# Autodesk Inventor assembly: componentStack
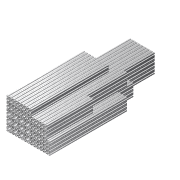
[picture p0: Inventor's stored thumbnail of the model, 180x180]
Saved by Autodesk Inventor 2018 (Build 220112000, 112)
## iProperties
Created: 2018-01-08
Part Number: componentStack
Document SubType Name: Assembly
Designer: sawaiz
Author: sawaiz
## Documents named in this file (7)
- C:\Users\sawaiz\OneDrive\personal\berlin\Move\larkspur\kitchen\frame\extrusions\componentStack.iam
- C:\Users\sawaiz\OneDrive\personal\berlin\Move\larkspur\kitchen\frame\extrusions\HFS5-4040-800.ipt
- C:\Users\sawaiz\OneDrive\personal\berlin\Move\larkspur\kitchen\frame\extrusions\HFS5-2040-500.ipt
- C:\Users\sawaiz\OneDrive\personal\berlin\Move\larkspur\kitchen\frame\extrusions\HFS5-2040-600.ipt
- C:\Users\sawaiz\OneDrive\personal\berlin\Move\larkspur\kitchen\frame\extrusions\HFS5-2020-500.ipt
- C:\Users\sawaiz\OneDrive\personal\berlin\Move\larkspur\kitchen\frame\extrusions\HFS5-2040-560.ipt
- C:\Users\sawaiz\OneDrive\personal\berlin\Move\larkspur\kitchen\frame\extrusions\HFS5-2040-300.ipt
## Components (56 placed, 6 different names)
1. HFS5-4040-800:1 — Flush:2, Mate:3, Flush:5, Flush:6
2. HFS5-4040-800:2
3. HFS5-4040-800:3 — Mate:1
4. HFS5-4040-800:4
5. HFS5-4040-800:5
6. HFS5-4040-800:6
7. HFS5-4040-800:7
8. HFS5-4040-800:8
9. HFS5-4040-800:9
10. HFS5-4040-800:10
11. HFS5-4040-800:11
12. HFS5-4040-800:12 — Flush:1
13. HFS5-2040-500:1 — Flush:1, Flush:2, Mate:5
14. HFS5-2040-500:2
15. HFS5-2040-500:3
16. HFS5-2040-500:4
17. HFS5-2040-500:5 — Mate:1
18. HFS5-2040-500:6
19. HFS5-2040-500:7
20. HFS5-2040-500:8
21. HFS5-2040-500:9
22. HFS5-2040-500:10
23. HFS5-2040-500:11
24. HFS5-2040-500:12
25. HFS5-2040-500:13
26. HFS5-2040-500:14
27. HFS5-2040-500:15
28. HFS5-2040-500:16
29. HFS5-2040-600:1 — Mate:3, Flush:6
30. HFS5-2040-600:2 — Mate:4
31. HFS5-2040-600:3 — Flush:5
32. HFS5-2040-600:4
33. HFS5-2040-600:5
34. HFS5-2040-600:6 — Mate:2, Flush:3, Flush:4
35. HFS5-2020-500:1
36. HFS5-2020-500:2
37. HFS5-2020-500:3 — Flush:4
38. HFS5-2020-500:4
39. HFS5-2020-500:5
40. HFS5-2020-500:6 — Flush:7
41. HFS5-2020-500:7
42. HFS5-2020-500:8
43. HFS5-2020-500:9 — Mate:2
44. HFS5-2020-500:10
45. HFS5-2020-500:11 — Flush:3
46. HFS5-2020-500:12
47. HFS5-2040-560:1 — Mate:4, Mate:6
48. HFS5-2040-560:2 — Flush:8, Flush:9
49. HFS5-2040-560:3
50. HFS5-2040-560:4
51. HFS5-2040-560:5 — Flush:7, Mate:5
52. HFS5-2040-560:6
53. HFS5-2040-300:1
54. HFS5-2040-300:2
55. HFS5-2040-300:3
56. HFS5-2040-300:4 — Mate:6, Flush:8, Flush:9
## Component patterns: (12 elements, first: HFS5-4040-800:1), (16 elements, first: HFS5-2040-500:1), (6 elements, first: HFS5-2040-600:1), (12 elements, first: HFS5-2020-500:1), (6 elements, first: HFS5-2040-560:1), (4 elements, first: HFS5-2040-300:1)
## Relationships (15: Flush 9, Mate 6)
- Flush:1: HFS5-4040-800:12 ↔ HFS5-2040-500:1
- Flush:2: HFS5-4040-800:1 ↔ HFS5-2040-500:1
- Mate:1: HFS5-4040-800:3 ↔ HFS5-2040-500:5
- Mate:2: HFS5-2040-600:6 ↔ HFS5-2020-500:9
- Flush:3: HFS5-2040-600:6 ↔ HFS5-2020-500:11
- Flush:4: HFS5-2040-600:6 ↔ HFS5-2020-500:3
- Mate:3: HFS5-4040-800:1 ↔ HFS5-2040-600:1
- Flush:5: HFS5-4040-800:1 ↔ HFS5-2040-600:3
- Flush:6: HFS5-4040-800:1 ↔ HFS5-2040-600:1
- Flush:7: HFS5-2020-500:6 ↔ HFS5-2040-560:5
- Mate:4: HFS5-2040-600:2 ↔ HFS5-2040-560:1
- Mate:5: HFS5-2040-500:1 ↔ HFS5-2040-560:5
- Mate:6: HFS5-2040-560:1 ↔ HFS5-2040-300:4
- Flush:8: HFS5-2040-560:2 ↔ HFS5-2040-300:4
- Flush:9: HFS5-2040-560:2 ↔ HFS5-2040-300:4
